# Autodesk Inventor assembly: basketball hoop
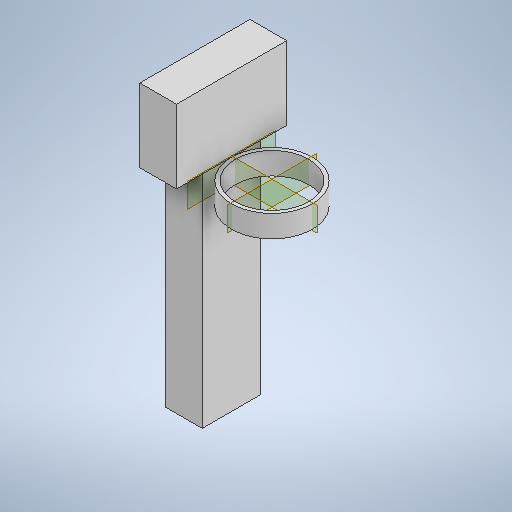
[picture p0: Inventor's stored thumbnail of the model, 512x512]
Saved by Autodesk Inventor 2026.1 (Build 301233020, 233B)
## iProperties
Created: 2026-01-04
Part Number: basketball hoop
Document SubType Name: Assembly
Designer: aa992
Author: aa992
## Documents named in this file (4)
- C:\Users\aa992\OneDrive\Desktop\basketball hoop.iam
- C:\Users\aa992\OneDrive\Desktop\backboard.ipt
- C:\Users\aa992\OneDrive\Desktop\basketball post.ipt
- C:\Users\aa992\OneDrive\Desktop\rim.ipt
## Components (3 placed, 3 different names)
1. backboard:1 — Mate:1, Flush:1, Flush:2, Mate:2, Flush:3, Flush:4
2. basketball post:1 — Mate:2, Flush:3, Flush:4, Mate:3, Mate:4, Mate:5
3. rim:1 — Mate:3, Mate:4, Mate:5
## Relationships (9: Mate 5, Flush 4)
- Mate:1: backboard:1
- Flush:1: backboard:1
- Flush:2: backboard:1
- Mate:2: backboard:1 ↔ basketball post:1
- Flush:3: backboard:1 ↔ basketball post:1
- Flush:4 (-35 mm): backboard:1 ↔ basketball post:1
- Mate:3: basketball post:1 ↔ rim:1
- Mate:4 (0.1 mm): basketball post:1 ↔ rim:1
- Mate:5 (0.1 mm): basketball post:1 ↔ rim:1
